# Autodesk Inventor assembly: still pipe
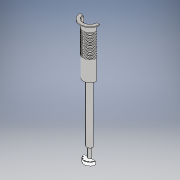
[picture p0: Inventor's stored thumbnail of the model, 180x180]
Saved by Autodesk Inventor 2018 (Build 220112000, 112)
## iProperties
Created: 2019-01-14
Part Number: still pipe
Document SubType Name: Assembly
Designer: Admin
Author: Admin
## Documents named in this file (6)
- C:\Users\freyja\Documents\Cryostat\CAD\still pipe.iam
- C:\Users\freyja\Documents\Cryostat\CAD\KF50 bellows.ipt
- C:\Users\freyja\Documents\Cryostat\CAD\still pipe small.iam.ipt
- C:\Users\freyja\Documents\Cryostat\CAD\universal connector.ipt
- C:\Users\freyja\Documents\Cryostat\CAD\weldpart.ipt
- still pipe small.iam
## Components (4 placed, 4 different names)
1. KF50 bellows:1 — Mate:1, Mate:3, Mate:4
2. still pipe small.iam:1 — Mate:1, Mate:2, Flush:1, Flush:2
3. universal connector:1 — Mate:2, Flush:1
4. weldpart:1 — Mate:3, Mate:4, Flush:2
## Relationships (6: Mate 4, Flush 2)
- Mate:1: KF50 bellows:1 ↔ still pipe small.iam:1
- Mate:2: still pipe small.iam:1 ↔ universal connector:1
- Flush:1: still pipe small.iam:1 ↔ universal connector:1
- Mate:3: KF50 bellows:1 ↔ weldpart:1
- Mate:4 (-3.81 mm): KF50 bellows:1 ↔ weldpart:1
- Flush:2 (-1.27 mm): still pipe small.iam:1 ↔ weldpart:1
